# Autodesk Inventor assembly: arm_assy_v2
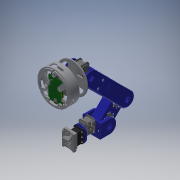
[picture p0: Inventor's stored thumbnail of the model, 180x180]
Saved by Autodesk Inventor 2018 (Build 220112000, 112)
## iProperties
Created: 2018-04-10
Part Number: arm_assy_v2
Document SubType Name: Assembly
Designer: mshaw2
Author: Matt Shaw
Title: Mk1 General Arrangement
## Documents named in this file (19)
- C:\Users\mshaw2\OneDrive - University of Plymouth\ROCO224\arm_assy_v2.iam
- C:\Users\mshaw2\OneDrive - University of Plymouth\ROCO224\arm_segment_1_2c.ipt
- C:\Users\mshaw2\OneDrive - University of Plymouth\ROCO224\arm_segment_2_1.ipt
- C:\Users\mshaw2\OneDrive - University of Plymouth\ROCO224\ENS_SERVO-RX-28.iam
- C:\Users\mshaw2\OneDrive - University of Plymouth\ROCO224\base_turret_v1.ipt
- C:\Users\mshaw2\OneDrive - University of Plymouth\ROCO224\arm_segment_1_1a.ipt
- C:\Users\mshaw2\OneDrive - University of Plymouth\ROCO224\arm_segment_1_1b.ipt
- C:\Users\mshaw2\OneDrive - University of Plymouth\ROCO224\grabber_rotating_mount_1.ipt
- C:\Users\mshaw2\OneDrive - University of Plymouth\ROCO224\Grabber_Assy.iam
- C:\Users\mshaw2\OneDrive - University of Plymouth\ROCO224\base_enclosure_1.ipt
- C:\Users\mshaw2\OneDrive - University of Plymouth\ROCO224\arm_segment_3_2a.ipt
- C:\Users\mshaw2\OneDrive - University of Plymouth\ROCO224\arm_segment_3_2b.ipt
- C:\Users\mshaw2\Documents\Inventor\Content Center Files\R2018\en-US\ISO 4762(2)\ISO 4762 - M6 x 25ISO.ipt
- C:\Users\mshaw2\Documents\Inventor\Content Center Files\R2018\en-US\SS-ISO 4762\ISO 4762 - M6 x 60SS-ISO.ipt
- C:\Users\mshaw2\Documents\Inventor\Content Center Files\R2018\en-US\ISO 4032(2)\ISO 4032 - M6 - ISO.ipt
- C:\Users\mshaw2\Documents\Inventor\Content Center Files\R2018\en-US\SS-ISO 4762\ISO 4762 - M2.5 x 8SS-ISO.ipt
- C:\Users\mshaw2\OneDrive - University of Plymouth\ROCO224\swivel_servo_cowl_1.ipt
- C:\Users\mshaw2\OneDrive - University of Plymouth\ROCO224\base_enclosure_2.ipt
- C:\Users\mshaw2\OneDrive - University of Plymouth\ROCO224\RPI3B+.ipt
## Components (70 placed, 18 different names)
1. arm_segment_1_2c:1 — Rigid:4, Rotational:2, Angle:4, Insert:4
2. arm_segment_2_1:1 — Rigid:6, Insert:25, Insert:26, Insert:27, Insert:28, Insert:29, Insert:30, Insert:31, Insert:32, Insert:33, Insert:34, Insert:35, Insert:36, Insert:37, Insert:38, Insert:39, Insert:40
3. ENS_SERVO-RX-28:1 [sub-assembly] — Rigid:5, Rigid:6, Rotational:2
4. arm_segment_1_2c:2 — Rigid:3, Insert:3
5. arm_segment_2_1:2 — Rigid:5, Rigid:7, Angle:3, Insert:9, Insert:10, Insert:11, Insert:12, Insert:13, Insert:14, Insert:15, Insert:16, Insert:17, Insert:18, Insert:19, Insert:20, Insert:21, Insert:22, Insert:23, Insert:24
6. ENS_SERVO-RX-28:2 [sub-assembly] — Rigid:1, Rotational:1
7. base_turret_v1:1 — Rigid:1, Angle:2, Rotational:5
8. arm_segment_1_1a:1 — Rigid:2, Rigid:3, Insert:5, Insert:6, Mate:4
9. arm_segment_1_1b:1 — Rigid:2, Rotational:1, Rigid:4, Angle:2, Angle:3, Mate:2, Insert:7, Insert:8, Angle:6, Angle:7
10. ENS_SERVO-RX-28:3 [sub-assembly] — Rotational:4, Rigid:11, Rigid:12
11. ENS_SERVO-RX-28:4 [sub-assembly] — Rigid:7, Rotational:7
12. grabber_rotating_mount_1:1 — Rotational:4, Rigid:9
13. Grabber_Assy:1 [sub-assembly] — Rigid:9, Insert:41, Insert:42, Insert:43, Insert:45, Insert:46, Insert:47
14. ENS_SERVO-RX-28:5 [sub-assembly] — Rotational:5, Rotational:6
15. base_enclosure_1:1 — Rotational:6, Rigid:13
16. arm_segment_3_2a:1 — Rigid:10, Angle:4, Mate:5, Mate:6, Mate:7, Mate:8, Mate:9, Mate:10, Mate:11, Mate:12, Rigid:11
17. arm_segment_3_2b:1 — Rigid:10, Rotational:7
18. swivel_servo_cowl_1:1 — Rigid:12
19. base_enclosure_2:1 — Rigid:13, Rigid:14
20. RPI3B+:1 — Rigid:14
21. ISO 4762 M6 x 25:1 — Insert:3, Mate:3
22. ISO 4762 M6 x 25:2 — Insert:4, Mate:1
23. SS ISO 4762 M6 x 60:1 — Insert:5
24. SS ISO 4762 M6 x 60:2 — Insert:6
25. ISO 4032 M6:1 — Mate:1, Mate:2
26. ISO 4032 M6:2 — Mate:3, Mate:4
27. ISO 4032 M6:3 — Insert:7, Angle:7
28. ISO 4032 M6:4 — Insert:8, Angle:6
29. SS ISO 4762 M2.5 x 8:1 — Insert:9
30. SS ISO 4762 M2.5 x 8:2 — Insert:10
31. SS ISO 4762 M2.5 x 8:3 — Insert:11
32. SS ISO 4762 M2.5 x 8:4 — Insert:12
33. SS ISO 4762 M2.5 x 8:5 — Insert:13
34. SS ISO 4762 M2.5 x 8:6 — Insert:14
35. SS ISO 4762 M2.5 x 8:7 — Insert:15
36. SS ISO 4762 M2.5 x 8:8 — Insert:16
37. SS ISO 4762 M2.5 x 8:9 — Insert:17
38. SS ISO 4762 M2.5 x 8:10 — Insert:18
39. SS ISO 4762 M2.5 x 8:11 — Insert:19
40. SS ISO 4762 M2.5 x 8:12 — Insert:20
41. SS ISO 4762 M2.5 x 8:13 — Insert:21
42. SS ISO 4762 M2.5 x 8:14 — Insert:22
43. SS ISO 4762 M2.5 x 8:15 — Insert:23
44. SS ISO 4762 M2.5 x 8:16 — Insert:24
45. SS ISO 4762 M2.5 x 8:17 — Insert:25
46. SS ISO 4762 M2.5 x 8:18 — Insert:26
47. SS ISO 4762 M2.5 x 8:19 — Insert:27
48. SS ISO 4762 M2.5 x 8:20 — Insert:28
49. SS ISO 4762 M2.5 x 8:21 — Insert:29
50. SS ISO 4762 M2.5 x 8:22 — Insert:30
51. SS ISO 4762 M2.5 x 8:23 — Insert:31
52. SS ISO 4762 M2.5 x 8:24 — Insert:32
53. SS ISO 4762 M2.5 x 8:25 — Insert:33
54. SS ISO 4762 M2.5 x 8:26 — Insert:34
55. SS ISO 4762 M2.5 x 8:27 — Insert:35
56. SS ISO 4762 M2.5 x 8:28 — Insert:36
57. SS ISO 4762 M2.5 x 8:29 — Insert:37
58. SS ISO 4762 M2.5 x 8:30 — Insert:38
59. SS ISO 4762 M2.5 x 8:31 — Insert:39
60. SS ISO 4762 M2.5 x 8:32 — Insert:40
61. SS ISO 4762 M2.5 x 8:33 — Insert:41
62. SS ISO 4762 M2.5 x 8:34 — Insert:42
63. SS ISO 4762 M2.5 x 8:35 — Insert:43
64. SS ISO 4762 M2.5 x 8:36 — Insert:45
65. SS ISO 4762 M2.5 x 8:37 — Insert:46
66. SS ISO 4762 M2.5 x 8:38 — Insert:47
67. SS ISO 4762 M2.5 x 8:39 — Mate:5, Mate:6
68. SS ISO 4762 M2.5 x 8:40 — Mate:7, Mate:8
69. SS ISO 4762 M2.5 x 8:41 — Mate:9, Mate:10
70. SS ISO 4762 M2.5 x 8:42 — Mate:11, Mate:12
## Relationships (80: Insert 44, WeldJoint 13, Mate 12, RevoluteJoint 6, Angle 5)
- Rigid:1 [WeldJoint]: ENS_SERVO-RX-28:2 ↔ base_turret_v1:1
- Rigid:2 [WeldJoint]: arm_segment_1_1a:1 ↔ arm_segment_1_1b:1
- Rotational:1 [RevoluteJoint] (0.5 mm): ENS_SERVO-RX-28:2 ↔ arm_segment_1_1b:1
- Rigid:3 [WeldJoint]: arm_segment_1_2c:2 ↔ arm_segment_1_1a:1
- Rigid:4 [WeldJoint]: arm_segment_1_2c:1 ↔ arm_segment_1_1b:1
- Rigid:5 [WeldJoint]: ENS_SERVO-RX-28:1 ↔ arm_segment_2_1:2
- Rigid:6 [WeldJoint]: arm_segment_2_1:1 ↔ ENS_SERVO-RX-28:1
- Rotational:2 [RevoluteJoint] (-0.5 mm): arm_segment_1_2c:1 ↔ ENS_SERVO-RX-28:1
- Rigid:7 [WeldJoint]: arm_segment_2_1:2 ↔ ENS_SERVO-RX-28:4
- Rotational:4 [RevoluteJoint]: ENS_SERVO-RX-28:3 ↔ grabber_rotating_mount_1:1
- Angle:2 (45 deg): base_turret_v1:1 ↔ arm_segment_1_1b:1
- Angle:3 (-90 deg): arm_segment_2_1:2 ↔ arm_segment_1_1b:1
- Rigid:9 [WeldJoint]: grabber_rotating_mount_1:1 ↔ Grabber_Assy:1
- Rotational:5 [RevoluteJoint]: base_turret_v1:1 ↔ ENS_SERVO-RX-28:5
- Rotational:6 [RevoluteJoint]: ENS_SERVO-RX-28:5 ↔ base_enclosure_1:1
- Rigid:10 [WeldJoint]: arm_segment_3_2a:1 ↔ arm_segment_3_2b:1
- Rotational:7 [RevoluteJoint] (0.5 mm): ENS_SERVO-RX-28:4 ↔ arm_segment_3_2b:1
- Angle:4 (45 deg): arm_segment_1_2c:1 ↔ arm_segment_3_2a:1
- Insert:3: arm_segment_1_2c:2 ↔ ISO 4762 M6 x 25:1
- Insert:4: arm_segment_1_2c:1 ↔ ISO 4762 M6 x 25:2
- Insert:5: arm_segment_1_1a:1 ↔ SS ISO 4762 M6 x 60:1
- Insert:6: arm_segment_1_1a:1 ↔ SS ISO 4762 M6 x 60:2
- Mate:1: ISO 4762 M6 x 25:2 ↔ ISO 4032 M6:1
- Mate:2: arm_segment_1_1b:1 ↔ ISO 4032 M6:1
- Mate:3: ISO 4762 M6 x 25:1 ↔ ISO 4032 M6:2
- Mate:4: arm_segment_1_1a:1 ↔ ISO 4032 M6:2
- Insert:7: arm_segment_1_1b:1 ↔ ISO 4032 M6:3
- Insert:8: arm_segment_1_1b:1 ↔ ISO 4032 M6:4
- Angle:6 (0 deg): arm_segment_1_1b:1 ↔ ISO 4032 M6:4
- Angle:7 (0 deg): arm_segment_1_1b:1 ↔ ISO 4032 M6:3
- Insert:9: arm_segment_2_1:2 ↔ SS ISO 4762 M2.5 x 8:1
- Insert:10: arm_segment_2_1:2 ↔ SS ISO 4762 M2.5 x 8:2
- Insert:11: arm_segment_2_1:2 ↔ SS ISO 4762 M2.5 x 8:3
- Insert:12: arm_segment_2_1:2 ↔ SS ISO 4762 M2.5 x 8:4
- Insert:13: arm_segment_2_1:2 ↔ SS ISO 4762 M2.5 x 8:5
- Insert:14: arm_segment_2_1:2 ↔ SS ISO 4762 M2.5 x 8:6
- Insert:15: arm_segment_2_1:2 ↔ SS ISO 4762 M2.5 x 8:7
- Insert:16: arm_segment_2_1:2 ↔ SS ISO 4762 M2.5 x 8:8
- Insert:17: arm_segment_2_1:2 ↔ SS ISO 4762 M2.5 x 8:9
- Insert:18: arm_segment_2_1:2 ↔ SS ISO 4762 M2.5 x 8:10
- Insert:19: arm_segment_2_1:2 ↔ SS ISO 4762 M2.5 x 8:11
- Insert:20: arm_segment_2_1:2 ↔ SS ISO 4762 M2.5 x 8:12
- Insert:21: arm_segment_2_1:2 ↔ SS ISO 4762 M2.5 x 8:13
- Insert:22: arm_segment_2_1:2 ↔ SS ISO 4762 M2.5 x 8:14
- Insert:23: arm_segment_2_1:2 ↔ SS ISO 4762 M2.5 x 8:15
- Insert:24: arm_segment_2_1:2 ↔ SS ISO 4762 M2.5 x 8:16
- Insert:25: arm_segment_2_1:1 ↔ SS ISO 4762 M2.5 x 8:17
- Insert:26: arm_segment_2_1:1 ↔ SS ISO 4762 M2.5 x 8:18
- Insert:27: arm_segment_2_1:1 ↔ SS ISO 4762 M2.5 x 8:19
- Insert:28: arm_segment_2_1:1 ↔ SS ISO 4762 M2.5 x 8:20
- Insert:29: arm_segment_2_1:1 ↔ SS ISO 4762 M2.5 x 8:21
- Insert:30: arm_segment_2_1:1 ↔ SS ISO 4762 M2.5 x 8:22
- Insert:31: arm_segment_2_1:1 ↔ SS ISO 4762 M2.5 x 8:23
- Insert:32: arm_segment_2_1:1 ↔ SS ISO 4762 M2.5 x 8:24
- Insert:33: arm_segment_2_1:1 ↔ SS ISO 4762 M2.5 x 8:25
- Insert:34: arm_segment_2_1:1 ↔ SS ISO 4762 M2.5 x 8:26
- Insert:35: arm_segment_2_1:1 ↔ SS ISO 4762 M2.5 x 8:27
- Insert:36: arm_segment_2_1:1 ↔ SS ISO 4762 M2.5 x 8:28
- Insert:37: arm_segment_2_1:1 ↔ SS ISO 4762 M2.5 x 8:29
- Insert:38: arm_segment_2_1:1 ↔ SS ISO 4762 M2.5 x 8:30
- Insert:39: arm_segment_2_1:1 ↔ SS ISO 4762 M2.5 x 8:31
- Insert:40: arm_segment_2_1:1 ↔ SS ISO 4762 M2.5 x 8:32
- Insert:41: Grabber_Assy:1 ↔ SS ISO 4762 M2.5 x 8:33
- Insert:42: Grabber_Assy:1 ↔ SS ISO 4762 M2.5 x 8:34
- Insert:43: Grabber_Assy:1 ↔ SS ISO 4762 M2.5 x 8:35
- Insert:45: Grabber_Assy:1 ↔ SS ISO 4762 M2.5 x 8:36
- Insert:46: Grabber_Assy:1 ↔ SS ISO 4762 M2.5 x 8:37
- Insert:47: Grabber_Assy:1 ↔ SS ISO 4762 M2.5 x 8:38
- Mate:5: arm_segment_3_2a:1 ↔ SS ISO 4762 M2.5 x 8:39
- Mate:6: arm_segment_3_2a:1 ↔ SS ISO 4762 M2.5 x 8:39
- Mate:7: arm_segment_3_2a:1 ↔ SS ISO 4762 M2.5 x 8:40
- Mate:8: arm_segment_3_2a:1 ↔ SS ISO 4762 M2.5 x 8:40
- Mate:9: arm_segment_3_2a:1 ↔ SS ISO 4762 M2.5 x 8:41
- Mate:10: arm_segment_3_2a:1 ↔ SS ISO 4762 M2.5 x 8:41
- Mate:11: arm_segment_3_2a:1 ↔ SS ISO 4762 M2.5 x 8:42
- Mate:12: arm_segment_3_2a:1 ↔ SS ISO 4762 M2.5 x 8:42
- Rigid:11 [WeldJoint]: ENS_SERVO-RX-28:3 ↔ arm_segment_3_2a:1
- Rigid:12 [WeldJoint]: ENS_SERVO-RX-28:3 ↔ swivel_servo_cowl_1:1
- Rigid:13 [WeldJoint]: base_enclosure_1:1 ↔ base_enclosure_2:1
- Rigid:14 [WeldJoint]: base_enclosure_2:1 ↔ RPI3B+:1
